# Autodesk Inventor assembly: Base_Teste
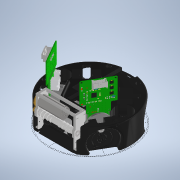
[picture p0: Inventor's stored thumbnail of the model, 180x180]
Saved by Autodesk Inventor 2020.2 (Build 242310000, 310)
## iProperties
Created: 2020-12-03
Part Number: Base_Teste
Document SubType Name: Assembly
Designer: Acer
Author: Acer
## Documents named in this file (6)
- C:\Users\Acer\Desktop\2020 LARC\2020_LARC\first_floor\Dribbler\Base_Teste.iam
- C:\Users\Acer\Desktop\2020 LARC\2020_LARC\first_floor\Base_RoboCIn.ipt
- C:\Users\Acer\Desktop\2020 LARC\2020_LARC\others\grass.ipt
- C:\Users\Acer\Desktop\2020 LARC\2020_LARC\first_floor\Dribbler\Dribbler.iam
- C:\Users\Acer\Desktop\2020 LARC\2020_LARC\first_floor\Motor\MaxonEC45-50W-MILE-Machined-with-gear.iam
- C:\Users\Acer\Desktop\2020 LARC\2020_LARC\kicker\kicker.iam
## Components (6 placed, 5 different names)
1. Base_RoboCIn:1 — Mate:1, Flush:1, Flush:2, Mate:3, Mate:4, Mate:6, Mate:7, Mate:8, Mate:9, Mate:10, Mate:11, Mate:12, Mate:13, Mate:14
2. grass:1 — Mate:1, Flush:1, Flush:2, Mate:5
3. Dribbler:1 [sub-assembly] — Mate:3, Mate:4, Mate:5
4. MG-MaxonEC45-50W-MILE:1 [sub-assembly] — Mate:6, Mate:10, Mate:11
5. MG-MaxonEC45-50W-MILE:2 [sub-assembly] — Mate:7, Mate:8, Mate:9
6. kicker:1 [sub-assembly] — Mate:12, Mate:13, Mate:14
## Relationships (15: Mate 13, Flush 2)
- Mate:1 (4.75 mm): Base_RoboCIn:1 ↔ grass:1
- Flush:1 (-200 mm): Base_RoboCIn:1 ↔ grass:1
- Flush:2 (-200 mm): Base_RoboCIn:1 ↔ grass:1
- Mate:3 (2 mm): Base_RoboCIn:1 ↔ Dribbler:1
- Mate:4 (1 mm): Base_RoboCIn:1 ↔ Dribbler:1
- Mate:5 (10 mm): grass:1 ↔ Dribbler:1
- Mate:6: Base_RoboCIn:1 ↔ MG-MaxonEC45-50W-MILE:1
- Mate:7: Base_RoboCIn:1 ↔ MG-MaxonEC45-50W-MILE:2
- Mate:8: Base_RoboCIn:1 ↔ MG-MaxonEC45-50W-MILE:2
- Mate:9: Base_RoboCIn:1 ↔ MG-MaxonEC45-50W-MILE:2
- Mate:10: Base_RoboCIn:1 ↔ MG-MaxonEC45-50W-MILE:1
- Mate:11: Base_RoboCIn:1 ↔ MG-MaxonEC45-50W-MILE:1
- Mate:12: Base_RoboCIn:1 ↔ kicker:1
- Mate:13: Base_RoboCIn:1 ↔ kicker:1
- Mate:14: Base_RoboCIn:1 ↔ kicker:1
